# Autodesk Inventor assembly: Drivetrain Side
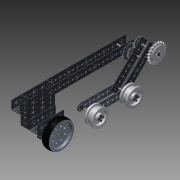
[picture p0: Inventor's stored thumbnail of the model, 180x180]
Saved by Autodesk Inventor 2015 (Build 190159000, 159)
## iProperties
Created: 2015-09-28
Part Number: Drivetrain Side
Document SubType Name: Assembly
Designer: Jing-Chen
Author: Jing-Chen
## Documents named in this file (8)
- C:\Users\Jing-Chen\Desktop\Bionic Hybrids 2016\Bionic-Hybrids\CAD\Drivetrain\Sub-Assemblies\Drivetrain Side.iam
- C:\Users\Jing-Chen\Desktop\Bionic Hybrids 2016\Bionic-Hybrids\Stock\Bracket-U25 - 739069.ipt
- C:\Users\Jing-Chen\Desktop\Bionic Hybrids 2016\Bionic-Hybrids\CAD\Drivetrain\Sub-Assemblies\Wheel Assembly.iam
- C:\Users\Jing-Chen\Desktop\Bionic Hybrids 2016\Bionic-Hybrids\CAD\Drivetrain\Sub-Assemblies\Track Frame Assembly.iam
- C:\Users\Jing-Chen\Desktop\Bionic Hybrids 2016\Bionic-Hybrids\Stock\Bearing-Thrust - 739091.ipt
- C:\Users\Jing-Chen\Desktop\Bionic Hybrids 2016\Bionic-Hybrids\Stock\Motor Mount - 739089.ipt
- C:\Users\Jing-Chen\Desktop\Bionic Hybrids 2016\Bionic-Hybrids\Stock\Bracket-U5 - 739066.ipt
- C:\Users\Jing-Chen\Desktop\Bionic Hybrids 2016\Bionic-Hybrids\CAD\Drivetrain\Modified Parts\Movable Motor.iam
## Components (9 placed, 7 different names)
1. Track Frame Assembly:1 [sub-assembly] — Mate:33, Mate:36
2. Bearing-Thrust - 739091:1 — Mate:33, Mate:34, Mate:35, Mate:36
3. Motor Mount - 739089:1 — Mate:40, Flush:1, Mate:51, Mate:52
4. Bracket-U25 - 739069:1 — Mate:34, Mate:35, Mate:42, Mate:43, Mate:45, Mate:48, Mate:49, Mate:50
5. Wheel Assembly:1 [sub-assembly] — Angle:2, Mate:41, Flush:2
6. Movable Motor:1 [sub-assembly] — Mate:40, Flush:1, Angle:1, Angle:2, Mate:41, Flush:2
7. Bracket-U5 - 739066:1 — Mate:44, Mate:46, Mate:47, Mate:51, Mate:52
8. Bracket-U5 - 739066:2 — Mate:42, Mate:43, Mate:44, Mate:45, Mate:46, Mate:47
9. Bracket-U5 - 739066:3 — Mate:48, Mate:49, Mate:50
## Relationships (21: Mate 17, Flush 2, Angle 2)
- Mate:33: Track Frame Assembly:1 ↔ Bearing-Thrust - 739091:1
- Mate:34: Bearing-Thrust - 739091:1 ↔ Bracket-U25 - 739069:1
- Mate:35: Bearing-Thrust - 739091:1 ↔ Bracket-U25 - 739069:1
- Mate:36: Track Frame Assembly:1 ↔ Bearing-Thrust - 739091:1
- Mate:40: Motor Mount - 739089:1 ↔ Movable Motor:1
- Flush:1: Motor Mount - 739089:1 ↔ Movable Motor:1
- Angle:1 (180 deg): Movable Motor:1
- Angle:2 (180 deg): Wheel Assembly:1 ↔ Movable Motor:1
- Mate:41: Wheel Assembly:1 ↔ Movable Motor:1
- Flush:2: Wheel Assembly:1 ↔ Movable Motor:1
- Mate:42: Bracket-U25 - 739069:1 ↔ Bracket-U5 - 739066:2
- Mate:43: Bracket-U25 - 739069:1 ↔ Bracket-U5 - 739066:2
- Mate:44: Bracket-U5 - 739066:1 ↔ Bracket-U5 - 739066:2
- Mate:45: Bracket-U25 - 739069:1 ↔ Bracket-U5 - 739066:2
- Mate:46: Bracket-U5 - 739066:1 ↔ Bracket-U5 - 739066:2
- Mate:47: Bracket-U5 - 739066:1 ↔ Bracket-U5 - 739066:2
- Mate:48: Bracket-U25 - 739069:1 ↔ Bracket-U5 - 739066:3
- Mate:49: Bracket-U25 - 739069:1 ↔ Bracket-U5 - 739066:3
- Mate:50: Bracket-U25 - 739069:1 ↔ Bracket-U5 - 739066:3
- Mate:51: Motor Mount - 739089:1 ↔ Bracket-U5 - 739066:1
- Mate:52: Motor Mount - 739089:1 ↔ Bracket-U5 - 739066:1
